(part 1 of 3)
# Autodesk Inventor assembly: coil_driver
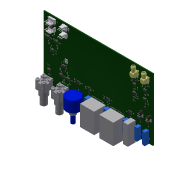
[picture p0: Inventor's stored thumbnail of the model, 180x180]
Saved by Autodesk Inventor 2017 (Build 210142000, 142)
## iProperties
Created: 2017-05-08
Part Number: coil_driver
Description: Component Model
Document SubType Name: Assembly
Designer: nfitch
Authority: Unknown
Sending System: Component
Preprocessor: Open CASCADE STEP processor 6.8
Title: C:/3D/sessions/PPP59106447bd5df/3d/Component/step_file.step
Author: Author
## Documents named in this file (964)
- C:\Users\nfitch\Desktop\repos\Imperial\CCMCircuits\CCM_0008_Coil_Driver\cad\coil_driver.iam
- C:\Users\nfitch\Desktop\repos\Imperial\CCMCircuits\CCM_0008_Coil_Driver\cad\RESC1608X056.ipt
- C:\Users\nfitch\Desktop\repos\Imperial\CCMCircuits\CCM_0008_Coil_Driver\cad\RESC1608X059.ipt
- C:\Users\nfitch\Desktop\repos\Imperial\CCMCircuits\CCM_0008_Coil_Driver\cad\RESC1608X057.ipt
- C:\Users\nfitch\Desktop\repos\Imperial\CCMCircuits\CCM_0008_Coil_Driver\cad\RESC1608X058.ipt
- C:\Users\nfitch\Desktop\repos\Imperial\CCMCircuits\CCM_0008_Coil_Driver\cad\RESC1608X55.ipt
- C:\Users\nfitch\Desktop\repos\Imperial\CCMCircuits\CCM_0008_Coil_Driver\cad\RESC1608X060.ipt
- C:\Users\nfitch\Desktop\repos\Imperial\CCMCircuits\CCM_0008_Coil_Driver\cad\RESC1608X061.ipt
- C:\Users\nfitch\Desktop\repos\Imperial\CCMCircuits\CCM_0008_Coil_Driver\cad\RESC1608X062.ipt
- C:\Users\nfitch\Desktop\repos\Imperial\CCMCircuits\CCM_0008_Coil_Driver\cad\RESC1608X063.ipt
- C:\Users\nfitch\Desktop\repos\Imperial\CCMCircuits\CCM_0008_Coil_Driver\cad\RESC1608X064.ipt
- C:\Users\nfitch\Desktop\repos\Imperial\CCMCircuits\CCM_0008_Coil_Driver\cad\RESC1608X065.ipt
- C:\Users\nfitch\Desktop\repos\Imperial\CCMCircuits\CCM_0008_Coil_Driver\cad\RESC1608X066.ipt
- C:\Users\nfitch\Desktop\repos\Imperial\CCMCircuits\CCM_0008_Coil_Driver\cad\RESC1608X067.ipt
- C:\Users\nfitch\Desktop\repos\Imperial\CCMCircuits\CCM_0008_Coil_Driver\cad\RESC1608X068.ipt
- C:\Users\nfitch\Desktop\repos\Imperial\CCMCircuits\CCM_0008_Coil_Driver\cad\RESC1608X069.ipt
- C:\Users\nfitch\Desktop\repos\Imperial\CCMCircuits\CCM_0008_Coil_Driver\cad\RESC1608X070.ipt
- C:\Users\nfitch\Desktop\repos\Imperial\CCMCircuits\CCM_0008_Coil_Driver\cad\RESC1608X071.ipt
- C:\Users\nfitch\Desktop\repos\Imperial\CCMCircuits\CCM_0008_Coil_Driver\cad\RESC1608X072.ipt
- C:\Users\nfitch\Desktop\repos\Imperial\CCMCircuits\CCM_0008_Coil_Driver\cad\RESC1608X073.ipt
- C:\Users\nfitch\Desktop\repos\Imperial\CCMCircuits\CCM_0008_Coil_Driver\cad\RESC1608X074.ipt
- C:\Users\nfitch\Desktop\repos\Imperial\CCMCircuits\CCM_0008_Coil_Driver\cad\RESC1608X075.ipt
- C:\Users\nfitch\Desktop\repos\Imperial\CCMCircuits\CCM_0008_Coil_Driver\cad\RESC1608X076.ipt
- C:\Users\nfitch\Desktop\repos\Imperial\CCMCircuits\CCM_0008_Coil_Driver\cad\RESC1608X077.ipt
- C:\Users\nfitch\Desktop\repos\Imperial\CCMCircuits\CCM_0008_Coil_Driver\cad\RESC1608X078.ipt
- C:\Users\nfitch\Desktop\repos\Imperial\CCMCircuits\CCM_0008_Coil_Driver\cad\RESC1608X079.ipt
- C:\Users\nfitch\Desktop\repos\Imperial\CCMCircuits\CCM_0008_Coil_Driver\cad\RESC1608X080.ipt
- C:\Users\nfitch\Desktop\repos\Imperial\CCMCircuits\CCM_0008_Coil_Driver\cad\RESC1608X081.ipt
- C:\Users\nfitch\Desktop\repos\Imperial\CCMCircuits\CCM_0008_Coil_Driver\cad\RESC1608X082.ipt
- C:\Users\nfitch\Desktop\repos\Imperial\CCMCircuits\CCM_0008_Coil_Driver\cad\RESC1608X083.ipt
- C:\Users\nfitch\Desktop\repos\Imperial\CCMCircuits\CCM_0008_Coil_Driver\cad\RESC1608X084.ipt
- C:\Users\nfitch\Desktop\repos\Imperial\CCMCircuits\CCM_0008_Coil_Driver\cad\RESC1608X085.ipt
- C:\Users\nfitch\Desktop\repos\Imperial\CCMCircuits\CCM_0008_Coil_Driver\cad\RESC1608X086.ipt
- C:\Users\nfitch\Desktop\repos\Imperial\CCMCircuits\CCM_0008_Coil_Driver\cad\RESC1608X087.ipt
- C:\Users\nfitch\Desktop\repos\Imperial\CCMCircuits\CCM_0008_Coil_Driver\cad\RESC1608X088.ipt
- C:\Users\nfitch\Desktop\repos\Imperial\CCMCircuits\CCM_0008_Coil_Driver\cad\RESC1608X089.ipt
- C:\Users\nfitch\Desktop\repos\Imperial\CCMCircuits\CCM_0008_Coil_Driver\cad\RESC1608X090.ipt
- C:\Users\nfitch\Desktop\repos\Imperial\CCMCircuits\CCM_0008_Coil_Driver\cad\RESC1608X091.ipt
- C:\Users\nfitch\Desktop\repos\Imperial\CCMCircuits\CCM_0008_Coil_Driver\cad\RESC1608X092.ipt
- C:\Users\nfitch\Desktop\repos\Imperial\CCMCircuits\CCM_0008_Coil_Driver\cad\RESC1608X093.ipt
- C:\Users\nfitch\Desktop\repos\Imperial\CCMCircuits\CCM_0008_Coil_Driver\cad\RESC1608X094.ipt
- C:\Users\nfitch\Desktop\repos\Imperial\CCMCircuits\CCM_0008_Coil_Driver\cad\RESC1608X095.ipt
- C:\Users\nfitch\Desktop\repos\Imperial\CCMCircuits\CCM_0008_Coil_Driver\cad\RESC1608X096.ipt
- C:\Users\nfitch\Desktop\repos\Imperial\CCMCircuits\CCM_0008_Coil_Driver\cad\RESC1608X097.ipt
- C:\Users\nfitch\Desktop\repos\Imperial\CCMCircuits\CCM_0008_Coil_Driver\cad\RESC1608X098.ipt
- C:\Users\nfitch\Desktop\repos\Imperial\CCMCircuits\CCM_0008_Coil_Driver\cad\RESC1608X099.ipt
- C:\Users\nfitch\Desktop\repos\Imperial\CCMCircuits\CCM_0008_Coil_Driver\cad\RESC1608X100.ipt
- C:\Users\nfitch\Desktop\repos\Imperial\CCMCircuits\CCM_0008_Coil_Driver\cad\RESC1608X101.ipt
- C:\Users\nfitch\Desktop\repos\Imperial\CCMCircuits\CCM_0008_Coil_Driver\cad\RESC1608X102.ipt
- C:\Users\nfitch\Desktop\repos\Imperial\CCMCircuits\CCM_0008_Coil_Driver\cad\RESC1608X103.ipt
- C:\Users\nfitch\Desktop\repos\Imperial\CCMCircuits\CCM_0008_Coil_Driver\cad\RESC1608X104.ipt
- C:\Users\nfitch\Desktop\repos\Imperial\CCMCircuits\CCM_0008_Coil_Driver\cad\RESC1608X105.ipt
- C:\Users\nfitch\Desktop\repos\Imperial\CCMCircuits\CCM_0008_Coil_Driver\cad\RESC1608X106.ipt
- C:\Users\nfitch\Desktop\repos\Imperial\CCMCircuits\CCM_0008_Coil_Driver\cad\RESC1608X107.ipt
- C:\Users\nfitch\Desktop\repos\Imperial\CCMCircuits\CCM_0008_Coil_Driver\cad\RESC1608X108.ipt
- C:\Users\nfitch\Desktop\repos\Imperial\CCMCircuits\CCM_0008_Coil_Driver\cad\RESC1608X109.ipt
- C:\Users\nfitch\Desktop\repos\Imperial\CCMCircuits\CCM_0008_Coil_Driver\cad\RESC1608X110.ipt
- C:\Users\nfitch\Desktop\repos\Imperial\CCMCircuits\CCM_0008_Coil_Driver\cad\RESC1608X111.ipt
- C:\Users\nfitch\Desktop\repos\Imperial\CCMCircuits\CCM_0008_Coil_Driver\cad\RESC1608X112.ipt
- C:\Users\nfitch\Desktop\repos\Imperial\CCMCircuits\CCM_0008_Coil_Driver\cad\RESC1608X113.ipt
- C:\Users\nfitch\Desktop\repos\Imperial\CCMCircuits\CCM_0008_Coil_Driver\cad\RESC1608X114.ipt
- C:\Users\nfitch\Desktop\repos\Imperial\CCMCircuits\CCM_0008_Coil_Driver\cad\RESC1608X115.ipt
- C:\Users\nfitch\Desktop\repos\Imperial\CCMCircuits\CCM_0008_Coil_Driver\cad\RESC1608X116.ipt
- C:\Users\nfitch\Desktop\repos\Imperial\CCMCircuits\CCM_0008_Coil_Driver\cad\RESC1608X117.ipt
- C:\Users\nfitch\Desktop\repos\Imperial\CCMCircuits\CCM_0008_Coil_Driver\cad\RESC1608X118.ipt
- C:\Users\nfitch\Desktop\repos\Imperial\CCMCircuits\CCM_0008_Coil_Driver\cad\RESC1608X119.ipt
- C:\Users\nfitch\Desktop\repos\Imperial\CCMCircuits\CCM_0008_Coil_Driver\cad\RESC1608X120.ipt
- C:\Users\nfitch\Desktop\repos\Imperial\CCMCircuits\CCM_0008_Coil_Driver\cad\RESC1608X121.ipt
- C:\Users\nfitch\Desktop\repos\Imperial\CCMCircuits\CCM_0008_Coil_Driver\cad\RESC1608X122.ipt
- C:\Users\nfitch\Desktop\repos\Imperial\CCMCircuits\CCM_0008_Coil_Driver\cad\RESC1608X123.ipt
- C:\Users\nfitch\Desktop\repos\Imperial\CCMCircuits\CCM_0008_Coil_Driver\cad\RESC1608X124.ipt
- C:\Users\nfitch\Desktop\repos\Imperial\CCMCircuits\CCM_0008_Coil_Driver\cad\RESC1608X125.ipt
- C:\Users\nfitch\Desktop\repos\Imperial\CCMCircuits\CCM_0008_Coil_Driver\cad\RESC1608X126.ipt
- C:\Users\nfitch\Desktop\repos\Imperial\CCMCircuits\CCM_0008_Coil_Driver\cad\RESC1608X127.ipt
- C:\Users\nfitch\Desktop\repos\Imperial\CCMCircuits\CCM_0008_Coil_Driver\cad\RESC1608X128.ipt
- C:\Users\nfitch\Desktop\repos\Imperial\CCMCircuits\CCM_0008_Coil_Driver\cad\RESC1608X129.ipt
- C:\Users\nfitch\Desktop\repos\Imperial\CCMCircuits\CCM_0008_Coil_Driver\cad\RESC1608X130.ipt
- C:\Users\nfitch\Desktop\repos\Imperial\CCMCircuits\CCM_0008_Coil_Driver\cad\RESC1608X131.ipt
- C:\Users\nfitch\Desktop\repos\Imperial\CCMCircuits\CCM_0008_Coil_Driver\cad\RESC1608X132.ipt
- C:\Users\nfitch\Desktop\repos\Imperial\CCMCircuits\CCM_0008_Coil_Driver\cad\RESC1608X133.ipt
- C:\Users\nfitch\Desktop\repos\Imperial\CCMCircuits\CCM_0008_Coil_Driver\cad\RESC1608X134.ipt
- C:\Users\nfitch\Desktop\repos\Imperial\CCMCircuits\CCM_0008_Coil_Driver\cad\RESC1608X135.ipt
- C:\Users\nfitch\Desktop\repos\Imperial\CCMCircuits\CCM_0008_Coil_Driver\cad\RESC1608X136.ipt
- C:\Users\nfitch\Desktop\repos\Imperial\CCMCircuits\CCM_0008_Coil_Driver\cad\RESC1608X137.ipt
- C:\Users\nfitch\Desktop\repos\Imperial\CCMCircuits\CCM_0008_Coil_Driver\cad\RESC1608X138.ipt
- C:\Users\nfitch\Desktop\repos\Imperial\CCMCircuits\CCM_0008_Coil_Driver\cad\RESC1608X139.ipt
- C:\Users\nfitch\Desktop\repos\Imperial\CCMCircuits\CCM_0008_Coil_Driver\cad\RESC1608X140.ipt
- C:\Users\nfitch\Desktop\repos\Imperial\CCMCircuits\CCM_0008_Coil_Driver\cad\RESC1608X141.ipt
- C:\Users\nfitch\Desktop\repos\Imperial\CCMCircuits\CCM_0008_Coil_Driver\cad\RESC1608X142.ipt
- C:\Users\nfitch\Desktop\repos\Imperial\CCMCircuits\CCM_0008_Coil_Driver\cad\RESC1608X143.ipt
- C:\Users\nfitch\Desktop\repos\Imperial\CCMCircuits\CCM_0008_Coil_Driver\cad\RESC1608X144.ipt
- C:\Users\nfitch\Desktop\repos\Imperial\CCMCircuits\CCM_0008_Coil_Driver\cad\RESC1608X145.ipt
- C:\Users\nfitch\Desktop\repos\Imperial\CCMCircuits\CCM_0008_Coil_Driver\cad\RESC1608X146.ipt
- C:\Users\nfitch\Desktop\repos\Imperial\CCMCircuits\CCM_0008_Coil_Driver\cad\RESC1608X147.ipt
- C:\Users\nfitch\Desktop\repos\Imperial\CCMCircuits\CCM_0008_Coil_Driver\cad\RESC1608X148.ipt
- C:\Users\nfitch\Desktop\repos\Imperial\CCMCircuits\CCM_0008_Coil_Driver\cad\RESC1608X149.ipt
- C:\Users\nfitch\Desktop\repos\Imperial\CCMCircuits\CCM_0008_Coil_Driver\cad\RESC1608X150.ipt
- C:\Users\nfitch\Desktop\repos\Imperial\CCMCircuits\CCM_0008_Coil_Driver\cad\RESC1608X151.ipt
- C:\Users\nfitch\Desktop\repos\Imperial\CCMCircuits\CCM_0008_Coil_Driver\cad\RESC1608X152.ipt
- C:\Users\nfitch\Desktop\repos\Imperial\CCMCircuits\CCM_0008_Coil_Driver\cad\RESC1608X153.ipt
- C:\Users\nfitch\Desktop\repos\Imperial\CCMCircuits\CCM_0008_Coil_Driver\cad\RESC1608X154.ipt
- C:\Users\nfitch\Desktop\repos\Imperial\CCMCircuits\CCM_0008_Coil_Driver\cad\RESC1608X155.ipt
- C:\Users\nfitch\Desktop\repos\Imperial\CCMCircuits\CCM_0008_Coil_Driver\cad\RESC1608X156.ipt
- C:\Users\nfitch\Desktop\repos\Imperial\CCMCircuits\CCM_0008_Coil_Driver\cad\RESC1608X157.ipt
- C:\Users\nfitch\Desktop\repos\Imperial\CCMCircuits\CCM_0008_Coil_Driver\cad\RESC1608X158.ipt
- C:\Users\nfitch\Desktop\repos\Imperial\CCMCircuits\CCM_0008_Coil_Driver\cad\RESC1608X159.ipt
- C:\Users\nfitch\Desktop\repos\Imperial\CCMCircuits\CCM_0008_Coil_Driver\cad\RESC1608X160.ipt
- C:\Users\nfitch\Desktop\repos\Imperial\CCMCircuits\CCM_0008_Coil_Driver\cad\RESC1608X161.ipt
- C:\Users\nfitch\Desktop\repos\Imperial\CCMCircuits\CCM_0008_Coil_Driver\cad\RESC1608X162.ipt
- C:\Users\nfitch\Desktop\repos\Imperial\CCMCircuits\CCM_0008_Coil_Driver\cad\RESC1608X163.ipt
- C:\Users\nfitch\Desktop\repos\Imperial\CCMCircuits\CCM_0008_Coil_Driver\cad\RESC1608X164.ipt
- C:\Users\nfitch\Desktop\repos\Imperial\CCMCircuits\CCM_0008_Coil_Driver\cad\RESC1608X165.ipt
- C:\Users\nfitch\Desktop\repos\Imperial\CCMCircuits\CCM_0008_Coil_Driver\cad\RESC1608X166.ipt
- C:\Users\nfitch\Desktop\repos\Imperial\CCMCircuits\CCM_0008_Coil_Driver\cad\RESC1608X167.ipt
- C:\Users\nfitch\Desktop\repos\Imperial\CCMCircuits\CCM_0008_Coil_Driver\cad\RESC1608X168.ipt
- C:\Users\nfitch\Desktop\repos\Imperial\CCMCircuits\CCM_0008_Coil_Driver\cad\RESC1608X169.ipt
- C:\Users\nfitch\Desktop\repos\Imperial\CCMCircuits\CCM_0008_Coil_Driver\cad\RESC1608X170.ipt
- C:\Users\nfitch\Desktop\repos\Imperial\CCMCircuits\CCM_0008_Coil_Driver\cad\RESC1608X171.ipt
- C:\Users\nfitch\Desktop\repos\Imperial\CCMCircuits\CCM_0008_Coil_Driver\cad\RESC1608X172.ipt
- C:\Users\nfitch\Desktop\repos\Imperial\CCMCircuits\CCM_0008_Coil_Driver\cad\RESC1608X173.ipt
- C:\Users\nfitch\Desktop\repos\Imperial\CCMCircuits\CCM_0008_Coil_Driver\cad\RESC1608X174.ipt
- C:\Users\nfitch\Desktop\repos\Imperial\CCMCircuits\CCM_0008_Coil_Driver\cad\RESC1608X175.ipt
- C:\Users\nfitch\Desktop\repos\Imperial\CCMCircuits\CCM_0008_Coil_Driver\cad\RESC1608X176.ipt
- C:\Users\nfitch\Desktop\repos\Imperial\CCMCircuits\CCM_0008_Coil_Driver\cad\RESC1608X177.ipt
- C:\Users\nfitch\Desktop\repos\Imperial\CCMCircuits\CCM_0008_Coil_Driver\cad\RESC1608X178.ipt
- C:\Users\nfitch\Desktop\repos\Imperial\CCMCircuits\CCM_0008_Coil_Driver\cad\RESC1608X179.ipt
- C:\Users\nfitch\Desktop\repos\Imperial\CCMCircuits\CCM_0008_Coil_Driver\cad\RESC1608X180.ipt
- C:\Users\nfitch\Desktop\repos\Imperial\CCMCircuits\CCM_0008_Coil_Driver\cad\RESC1608X181.ipt
- C:\Users\nfitch\Desktop\repos\Imperial\CCMCircuits\CCM_0008_Coil_Driver\cad\RESC1608X182.ipt
- C:\Users\nfitch\Desktop\repos\Imperial\CCMCircuits\CCM_0008_Coil_Driver\cad\RESC1608X183.ipt
- C:\Users\nfitch\Desktop\repos\Imperial\CCMCircuits\CCM_0008_Coil_Driver\cad\RESC1608X184.ipt
- C:\Users\nfitch\Desktop\repos\Imperial\CCMCircuits\CCM_0008_Coil_Driver\cad\RESC1608X185.ipt
- C:\Users\nfitch\Desktop\repos\Imperial\CCMCircuits\CCM_0008_Coil_Driver\cad\RESC1608X186.ipt
- C:\Users\nfitch\Desktop\repos\Imperial\CCMCircuits\CCM_0008_Coil_Driver\cad\RESC1608X187.ipt
- C:\Users\nfitch\Desktop\repos\Imperial\CCMCircuits\CCM_0008_Coil_Driver\cad\RESC1608X188.ipt
- C:\Users\nfitch\Desktop\repos\Imperial\CCMCircuits\CCM_0008_Coil_Driver\cad\RESC1608X189.ipt
- C:\Users\nfitch\Desktop\repos\Imperial\CCMCircuits\CCM_0008_Coil_Driver\cad\RESC1608X190.ipt
- C:\Users\nfitch\Desktop\repos\Imperial\CCMCircuits\CCM_0008_Coil_Driver\cad\RESC1608X191.ipt
- C:\Users\nfitch\Desktop\repos\Imperial\CCMCircuits\CCM_0008_Coil_Driver\cad\RESC1608X192.ipt
- C:\Users\nfitch\Desktop\repos\Imperial\CCMCircuits\CCM_0008_Coil_Driver\cad\RESC1608X193.ipt
- C:\Users\nfitch\Desktop\repos\Imperial\CCMCircuits\CCM_0008_Coil_Driver\cad\RESC1608X194.ipt
- C:\Users\nfitch\Desktop\repos\Imperial\CCMCircuits\CCM_0008_Coil_Driver\cad\RESC1608X195.ipt
- C:\Users\nfitch\Desktop\repos\Imperial\CCMCircuits\CCM_0008_Coil_Driver\cad\RESC1608X196.ipt
- C:\Users\nfitch\Desktop\repos\Imperial\CCMCircuits\CCM_0008_Coil_Driver\cad\RESC1608X197.ipt
- C:\Users\nfitch\Desktop\repos\Imperial\CCMCircuits\CCM_0008_Coil_Driver\cad\RESC1608X198.ipt
- C:\Users\nfitch\Desktop\repos\Imperial\CCMCircuits\CCM_0008_Coil_Driver\cad\RESC1608X199.ipt
- C:\Users\nfitch\Desktop\repos\Imperial\CCMCircuits\CCM_0008_Coil_Driver\cad\RESC1608X200.ipt
- C:\Users\nfitch\Desktop\repos\Imperial\CCMCircuits\CCM_0008_Coil_Driver\cad\RESC1608X201.ipt
- C:\Users\nfitch\Desktop\repos\Imperial\CCMCircuits\CCM_0008_Coil_Driver\cad\RESC1608X202.ipt
- C:\Users\nfitch\Desktop\repos\Imperial\CCMCircuits\CCM_0008_Coil_Driver\cad\RESC1608X203.ipt
- C:\Users\nfitch\Desktop\repos\Imperial\CCMCircuits\CCM_0008_Coil_Driver\cad\RESC1608X204.ipt
- C:\Users\nfitch\Desktop\repos\Imperial\CCMCircuits\CCM_0008_Coil_Driver\cad\RESC1608X205.ipt
- C:\Users\nfitch\Desktop\repos\Imperial\CCMCircuits\CCM_0008_Coil_Driver\cad\RESC1608X206.ipt
- C:\Users\nfitch\Desktop\repos\Imperial\CCMCircuits\CCM_0008_Coil_Driver\cad\RESC1608X207.ipt
- C:\Users\nfitch\Desktop\repos\Imperial\CCMCircuits\CCM_0008_Coil_Driver\cad\RESC1608X208.ipt
- C:\Users\nfitch\Desktop\repos\Imperial\CCMCircuits\CCM_0008_Coil_Driver\cad\RESC1608X209.ipt
- C:\Users\nfitch\Desktop\repos\Imperial\CCMCircuits\CCM_0008_Coil_Driver\cad\RESC1608X210.ipt
- C:\Users\nfitch\Desktop\repos\Imperial\CCMCircuits\CCM_0008_Coil_Driver\cad\RESC1608X211.ipt
- C:\Users\nfitch\Desktop\repos\Imperial\CCMCircuits\CCM_0008_Coil_Driver\cad\RESC1608X212.ipt
- C:\Users\nfitch\Desktop\repos\Imperial\CCMCircuits\CCM_0008_Coil_Driver\cad\RESC1608X213.ipt
- C:\Users\nfitch\Desktop\repos\Imperial\CCMCircuits\CCM_0008_Coil_Driver\cad\RESC1608X214.ipt
- C:\Users\nfitch\Desktop\repos\Imperial\CCMCircuits\CCM_0008_Coil_Driver\cad\RESC1608X215.ipt
- C:\Users\nfitch\Desktop\repos\Imperial\CCMCircuits\CCM_0008_Coil_Driver\cad\RESC1608X216.ipt
- C:\Users\nfitch\Desktop\repos\Imperial\CCMCircuits\CCM_0008_Coil_Driver\cad\RESC1608X217.ipt
- C:\Users\nfitch\Desktop\repos\Imperial\CCMCircuits\CCM_0008_Coil_Driver\cad\RESC1608X218.ipt
- C:\Users\nfitch\Desktop\repos\Imperial\CCMCircuits\CCM_0008_Coil_Driver\cad\RESC1608X219.ipt
- C:\Users\nfitch\Desktop\repos\Imperial\CCMCircuits\CCM_0008_Coil_Driver\cad\RESC1608X220.ipt
- C:\Users\nfitch\Desktop\repos\Imperial\CCMCircuits\CCM_0008_Coil_Driver\cad\RESC1608X221.ipt
- C:\Users\nfitch\Desktop\repos\Imperial\CCMCircuits\CCM_0008_Coil_Driver\cad\RESC1608X222.ipt
- C:\Users\nfitch\Desktop\repos\Imperial\CCMCircuits\CCM_0008_Coil_Driver\cad\RESC1608X223.ipt
- C:\Users\nfitch\Desktop\repos\Imperial\CCMCircuits\CCM_0008_Coil_Driver\cad\RESC1608X224.ipt
- C:\Users\nfitch\Desktop\repos\Imperial\CCMCircuits\CCM_0008_Coil_Driver\cad\RESC1608X225.ipt
- C:\Users\nfitch\Desktop\repos\Imperial\CCMCircuits\CCM_0008_Coil_Driver\cad\RESC1608X226.ipt
- C:\Users\nfitch\Desktop\repos\Imperial\CCMCircuits\CCM_0008_Coil_Driver\cad\RESC1608X227.ipt
- C:\Users\nfitch\Desktop\repos\Imperial\CCMCircuits\CCM_0008_Coil_Driver\cad\RESC1608X228.ipt
- C:\Users\nfitch\Desktop\repos\Imperial\CCMCircuits\CCM_0008_Coil_Driver\cad\RESC1608X229.ipt
- C:\Users\nfitch\Desktop\repos\Imperial\CCMCircuits\CCM_0008_Coil_Driver\cad\RESC1608X230.ipt
- C:\Users\nfitch\Desktop\repos\Imperial\CCMCircuits\CCM_0008_Coil_Driver\cad\RESC1608X231.ipt
- C:\Users\nfitch\Desktop\repos\Imperial\CCMCircuits\CCM_0008_Coil_Driver\cad\RESC1608X232.ipt
- C:\Users\nfitch\Desktop\repos\Imperial\CCMCircuits\CCM_0008_Coil_Driver\cad\RESC1608X233.ipt
- C:\Users\nfitch\Desktop\repos\Imperial\CCMCircuits\CCM_0008_Coil_Driver\cad\RESC1608X234.ipt
- C:\Users\nfitch\Desktop\repos\Imperial\CCMCircuits\CCM_0008_Coil_Driver\cad\RESC1608X235.ipt
- C:\Users\nfitch\Desktop\repos\Imperial\CCMCircuits\CCM_0008_Coil_Driver\cad\RESC1608X236.ipt
- C:\Users\nfitch\Desktop\repos\Imperial\CCMCircuits\CCM_0008_Coil_Driver\cad\RESC1608X237.ipt
- C:\Users\nfitch\Desktop\repos\Imperial\CCMCircuits\CCM_0008_Coil_Driver\cad\RESC1608X238.ipt
- C:\Users\nfitch\Desktop\repos\Imperial\CCMCircuits\CCM_0008_Coil_Driver\cad\RESC1608X239.ipt
- C:\Users\nfitch\Desktop\repos\Imperial\CCMCircuits\CCM_0008_Coil_Driver\cad\RESC1608X240.ipt
- C:\Users\nfitch\Desktop\repos\Imperial\CCMCircuits\CCM_0008_Coil_Driver\cad\RESC1608X241.ipt
- C:\Users\nfitch\Desktop\repos\Imperial\CCMCircuits\CCM_0008_Coil_Driver\cad\RESC1608X242.ipt
- C:\Users\nfitch\Desktop\repos\Imperial\CCMCircuits\CCM_0008_Coil_Driver\cad\RESC1608X243.ipt
- C:\Users\nfitch\Desktop\repos\Imperial\CCMCircuits\CCM_0008_Coil_Driver\cad\RESC1608X244.ipt
- C:\Users\nfitch\Desktop\repos\Imperial\CCMCircuits\CCM_0008_Coil_Driver\cad\RESC1608X245.ipt
- C:\Users\nfitch\Desktop\repos\Imperial\CCMCircuits\CCM_0008_Coil_Driver\cad\RESC1608X246.ipt
- C:\Users\nfitch\Desktop\repos\Imperial\CCMCircuits\CCM_0008_Coil_Driver\cad\RESC1608X247.ipt
- C:\Users\nfitch\Desktop\repos\Imperial\CCMCircuits\CCM_0008_Coil_Driver\cad\RESC1608X248.ipt
- C:\Users\nfitch\Desktop\repos\Imperial\CCMCircuits\CCM_0008_Coil_Driver\cad\RESC1608X249.ipt
- C:\Users\nfitch\Desktop\repos\Imperial\CCMCircuits\CCM_0008_Coil_Driver\cad\RESC1608X250.ipt
- C:\Users\nfitch\Desktop\repos\Imperial\CCMCircuits\CCM_0008_Coil_Driver\cad\RESC1608X251.ipt
- C:\Users\nfitch\Desktop\repos\Imperial\CCMCircuits\CCM_0008_Coil_Driver\cad\RESC1608X252.ipt
- C:\Users\nfitch\Desktop\repos\Imperial\CCMCircuits\CCM_0008_Coil_Driver\cad\RESC1608X253.ipt
- C:\Users\nfitch\Desktop\repos\Imperial\CCMCircuits\CCM_0008_Coil_Driver\cad\RESC1608X254.ipt
- C:\Users\nfitch\Desktop\repos\Imperial\CCMCircuits\CCM_0008_Coil_Driver\cad\RESC1608X255.ipt
- C:\Users\nfitch\Desktop\repos\Imperial\CCMCircuits\CCM_0008_Coil_Driver\cad\RESC1608X256.ipt
- C:\Users\nfitch\Desktop\repos\Imperial\CCMCircuits\CCM_0008_Coil_Driver\cad\RESC1608X257.ipt
- C:\Users\nfitch\Desktop\repos\Imperial\CCMCircuits\CCM_0008_Coil_Driver\cad\RESC1608X258.ipt
- C:\Users\nfitch\Desktop\repos\Imperial\CCMCircuits\CCM_0008_Coil_Driver\cad\RESC1608X259.ipt
- C:\Users\nfitch\Desktop\repos\Imperial\CCMCircuits\CCM_0008_Coil_Driver\cad\RESC1608X260.ipt
- C:\Users\nfitch\Desktop\repos\Imperial\CCMCircuits\CCM_0008_Coil_Driver\cad\RESC1608X261.ipt
- C:\Users\nfitch\Desktop\repos\Imperial\CCMCircuits\CCM_0008_Coil_Driver\cad\RESC1608X262.ipt
- C:\Users\nfitch\Desktop\repos\Imperial\CCMCircuits\CCM_0008_Coil_Driver\cad\RESC1608X263.ipt
- C:\Users\nfitch\Desktop\repos\Imperial\CCMCircuits\CCM_0008_Coil_Driver\cad\RESC1608X264.ipt
- C:\Users\nfitch\Desktop\repos\Imperial\CCMCircuits\CCM_0008_Coil_Driver\cad\RESC1608X265.ipt
- C:\Users\nfitch\Desktop\repos\Imperial\CCMCircuits\CCM_0008_Coil_Driver\cad\RESC1608X266.ipt
- C:\Users\nfitch\Desktop\repos\Imperial\CCMCircuits\CCM_0008_Coil_Driver\cad\RESC1608X267.ipt
- C:\Users\nfitch\Desktop\repos\Imperial\CCMCircuits\CCM_0008_Coil_Driver\cad\RESC1608X268.ipt
- C:\Users\nfitch\Desktop\repos\Imperial\CCMCircuits\CCM_0008_Coil_Driver\cad\RESC1608X269.ipt
- C:\Users\nfitch\Desktop\repos\Imperial\CCMCircuits\CCM_0008_Coil_Driver\cad\RESC1608X270.ipt
- C:\Users\nfitch\Desktop\repos\Imperial\CCMCircuits\CCM_0008_Coil_Driver\cad\RESC1608X271.ipt
- C:\Users\nfitch\Desktop\repos\Imperial\CCMCircuits\CCM_0008_Coil_Driver\cad\RESC1608X272.ipt
- C:\Users\nfitch\Desktop\repos\Imperial\CCMCircuits\CCM_0008_Coil_Driver\cad\RESC1608X273.ipt
- C:\Users\nfitch\Desktop\repos\Imperial\CCMCircuits\CCM_0008_Coil_Driver\cad\RESC1608X274.ipt
- C:\Users\nfitch\Desktop\repos\Imperial\CCMCircuits\CCM_0008_Coil_Driver\cad\RESC1608X275.ipt
- C:\Users\nfitch\Desktop\repos\Imperial\CCMCircuits\CCM_0008_Coil_Driver\cad\RESC1608X276.ipt
- C:\Users\nfitch\Desktop\repos\Imperial\CCMCircuits\CCM_0008_Coil_Driver\cad\RESC1608X277.ipt
- C:\Users\nfitch\Desktop\repos\Imperial\CCMCircuits\CCM_0008_Coil_Driver\cad\RESC1608X278.ipt
- C:\Users\nfitch\Desktop\repos\Imperial\CCMCircuits\CCM_0008_Coil_Driver\cad\RESC1608X279.ipt
- C:\Users\nfitch\Desktop\repos\Imperial\CCMCircuits\CCM_0008_Coil_Driver\cad\RESC1608X280.ipt
- C:\Users\nfitch\Desktop\repos\Imperial\CCMCircuits\CCM_0008_Coil_Driver\cad\RESC1608X281.ipt
- C:\Users\nfitch\Desktop\repos\Imperial\CCMCircuits\CCM_0008_Coil_Driver\cad\RESC1608X282.ipt
- C:\Users\nfitch\Desktop\repos\Imperial\CCMCircuits\CCM_0008_Coil_Driver\cad\RESC1608X283.ipt
- C:\Users\nfitch\Desktop\repos\Imperial\CCMCircuits\CCM_0008_Coil_Driver\cad\RESC1608X284.ipt
- C:\Users\nfitch\Desktop\repos\Imperial\CCMCircuits\CCM_0008_Coil_Driver\cad\RESC1608X285.ipt
- C:\Users\nfitch\Desktop\repos\Imperial\CCMCircuits\CCM_0008_Coil_Driver\cad\RESC1608X286.ipt
- C:\Users\nfitch\Desktop\repos\Imperial\CCMCircuits\CCM_0008_Coil_Driver\cad\RESC1608X287.ipt
- C:\Users\nfitch\Desktop\repos\Imperial\CCMCircuits\CCM_0008_Coil_Driver\cad\RESC1608X288.ipt
- C:\Users\nfitch\Desktop\repos\Imperial\CCMCircuits\CCM_0008_Coil_Driver\cad\RESC1608X289.ipt
- C:\Users\nfitch\Desktop\repos\Imperial\CCMCircuits\CCM_0008_Coil_Driver\cad\RESC1608X290.ipt
- C:\Users\nfitch\Desktop\repos\Imperial\CCMCircuits\CCM_0008_Coil_Driver\cad\RESC1608X291.ipt
- C:\Users\nfitch\Desktop\repos\Imperial\CCMCircuits\CCM_0008_Coil_Driver\cad\RESC1608X292.ipt
- C:\Users\nfitch\Desktop\repos\Imperial\CCMCircuits\CCM_0008_Coil_Driver\cad\RESC1608X293.ipt
- C:\Users\nfitch\Desktop\repos\Imperial\CCMCircuits\CCM_0008_Coil_Driver\cad\RESC1608X294.ipt
- C:\Users\nfitch\Desktop\repos\Imperial\CCMCircuits\CCM_0008_Coil_Driver\cad\RESC1608X295.ipt
- C:\Users\nfitch\Desktop\repos\Imperial\CCMCircuits\CCM_0008_Coil_Driver\cad\RESC1608X296.ipt
- C:\Users\nfitch\Desktop\repos\Imperial\CCMCircuits\CCM_0008_Coil_Driver\cad\RESC1608X297.ipt
- C:\Users\nfitch\Desktop\repos\Imperial\CCMCircuits\CCM_0008_Coil_Driver\cad\RESC1608X298.ipt
- C:\Users\nfitch\Desktop\repos\Imperial\CCMCircuits\CCM_0008_Coil_Driver\cad\RESC1608X299.ipt
- C:\Users\nfitch\Desktop\repos\Imperial\CCMCircuits\CCM_0008_Coil_Driver\cad\RESC1608X300.ipt
- C:\Users\nfitch\Desktop\repos\Imperial\CCMCircuits\CCM_0008_Coil_Driver\cad\RESC1608X301.ipt
- C:\Users\nfitch\Desktop\repos\Imperial\CCMCircuits\CCM_0008_Coil_Driver\cad\RESC1608X302.ipt
- C:\Users\nfitch\Desktop\repos\Imperial\CCMCircuits\CCM_0008_Coil_Driver\cad\RESC1608X303.ipt
- C:\Users\nfitch\Desktop\repos\Imperial\CCMCircuits\CCM_0008_Coil_Driver\cad\RESC1608X304.ipt
- C:\Users\nfitch\Desktop\repos\Imperial\CCMCircuits\CCM_0008_Coil_Driver\cad\RESC1608X305.ipt
- C:\Users\nfitch\Desktop\repos\Imperial\CCMCircuits\CCM_0008_Coil_Driver\cad\RESC1608X306.ipt
- C:\Users\nfitch\Desktop\repos\Imperial\CCMCircuits\CCM_0008_Coil_Driver\cad\RESC1608X307.ipt
- C:\Users\nfitch\Desktop\repos\Imperial\CCMCircuits\CCM_0008_Coil_Driver\cad\RESC1608X308.ipt
- C:\Users\nfitch\Desktop\repos\Imperial\CCMCircuits\CCM_0008_Coil_Driver\cad\RESC1608X309.ipt
- C:\Users\nfitch\Desktop\repos\Imperial\CCMCircuits\CCM_0008_Coil_Driver\cad\RESC1608X310.ipt
- C:\Users\nfitch\Desktop\repos\Imperial\CCMCircuits\CCM_0008_Coil_Driver\cad\RESC1608X311.ipt
- C:\Users\nfitch\Desktop\repos\Imperial\CCMCircuits\CCM_0008_Coil_Driver\cad\RESC1608X312.ipt
- C:\Users\nfitch\Desktop\repos\Imperial\CCMCircuits\CCM_0008_Coil_Driver\cad\RESC1608X313.ipt
- C:\Users\nfitch\Desktop\repos\Imperial\CCMCircuits\CCM_0008_Coil_Driver\cad\RESC1608X314.ipt
- C:\Users\nfitch\Desktop\repos\Imperial\CCMCircuits\CCM_0008_Coil_Driver\cad\RESC1608X315.ipt
- C:\Users\nfitch\Desktop\repos\Imperial\CCMCircuits\CCM_0008_Coil_Driver\cad\RESC1608X316.ipt
- C:\Users\nfitch\Desktop\repos\Imperial\CCMCircuits\CCM_0008_Coil_Driver\cad\RESC1608X317.ipt
- C:\Users\nfitch\Desktop\repos\Imperial\CCMCircuits\CCM_0008_Coil_Driver\cad\RESC1608X318.ipt
- C:\Users\nfitch\Desktop\repos\Imperial\CCMCircuits\CCM_0008_Coil_Driver\cad\RESC1608X319.ipt
- C:\Users\nfitch\Desktop\repos\Imperial\CCMCircuits\CCM_0008_Coil_Driver\cad\RESC1608X320.ipt
- C:\Users\nfitch\Desktop\repos\Imperial\CCMCircuits\CCM_0008_Coil_Driver\cad\RESC1608X321.ipt
- C:\Users\nfitch\Desktop\repos\Imperial\CCMCircuits\CCM_0008_Coil_Driver\cad\RESC1608X322.ipt
- C:\Users\nfitch\Desktop\repos\Imperial\CCMCircuits\CCM_0008_Coil_Driver\cad\RESC1608X323.ipt
- C:\Users\nfitch\Desktop\repos\Imperial\CCMCircuits\CCM_0008_Coil_Driver\cad\RESC1608X324.ipt
- C:\Users\nfitch\Desktop\repos\Imperial\CCMCircuits\CCM_0008_Coil_Driver\cad\RESC1608X325.ipt
- C:\Users\nfitch\Desktop\repos\Imperial\CCMCircuits\CCM_0008_Coil_Driver\cad\RESC1608X326.ipt
- C:\Users\nfitch\Desktop\repos\Imperial\CCMCircuits\CCM_0008_Coil_Driver\cad\RESC1608X327.ipt
- C:\Users\nfitch\Desktop\repos\Imperial\CCMCircuits\CCM_0008_Coil_Driver\cad\RESC1608X328.ipt
- C:\Users\nfitch\Desktop\repos\Imperial\CCMCircuits\CCM_0008_Coil_Driver\cad\RESC1608X329.ipt
- C:\Users\nfitch\Desktop\repos\Imperial\CCMCircuits\CCM_0008_Coil_Driver\cad\RESC1608X330.ipt
- C:\Users\nfitch\Desktop\repos\Imperial\CCMCircuits\CCM_0008_Coil_Driver\cad\RESC1608X331.ipt
- C:\Users\nfitch\Desktop\repos\Imperial\CCMCircuits\CCM_0008_Coil_Driver\cad\RESC1608X332.ipt
- C:\Users\nfitch\Desktop\repos\Imperial\CCMCircuits\CCM_0008_Coil_Driver\cad\RESC1608X333.ipt
- C:\Users\nfitch\Desktop\repos\Imperial\CCMCircuits\CCM_0008_Coil_Driver\cad\RESC1608X334.ipt
- C:\Users\nfitch\Desktop\repos\Imperial\CCMCircuits\CCM_0008_Coil_Driver\cad\RESC1608X335.ipt
- C:\Users\nfitch\Desktop\repos\Imperial\CCMCircuits\CCM_0008_Coil_Driver\cad\RESC1608X336.ipt
- C:\Users\nfitch\Desktop\repos\Imperial\CCMCircuits\CCM_0008_Coil_Driver\cad\RESC1608X337.ipt
- C:\Users\nfitch\Desktop\repos\Imperial\CCMCircuits\CCM_0008_Coil_Driver\cad\RESC1608X338.ipt
- C:\Users\nfitch\Desktop\repos\Imperial\CCMCircuits\CCM_0008_Coil_Driver\cad\RESC1608X339.ipt
- C:\Users\nfitch\Desktop\repos\Imperial\CCMCircuits\CCM_0008_Coil_Driver\cad\RESC1608X340.ipt
- C:\Users\nfitch\Desktop\repos\Imperial\CCMCircuits\CCM_0008_Coil_Driver\cad\RESC1608X341.ipt
- C:\Users\nfitch\Desktop\repos\Imperial\CCMCircuits\CCM_0008_Coil_Driver\cad\RESC1608X342.ipt
- C:\Users\nfitch\Desktop\repos\Imperial\CCMCircuits\CCM_0008_Coil_Driver\cad\RESC1608X343.ipt
- C:\Users\nfitch\Desktop\repos\Imperial\CCMCircuits\CCM_0008_Coil_Driver\cad\RESC1608X344.ipt
- C:\Users\nfitch\Desktop\repos\Imperial\CCMCircuits\CCM_0008_Coil_Driver\cad\RESC1608X345.ipt
- C:\Users\nfitch\Desktop\repos\Imperial\CCMCircuits\CCM_0008_Coil_Driver\cad\RESC1608X346.ipt
- C:\Users\nfitch\Desktop\repos\Imperial\CCMCircuits\CCM_0008_Coil_Driver\cad\RESC1608X347.ipt
- C:\Users\nfitch\Desktop\repos\Imperial\CCMCircuits\CCM_0008_Coil_Driver\cad\RESC1608X348.ipt
- C:\Users\nfitch\Desktop\repos\Imperial\CCMCircuits\CCM_0008_Coil_Driver\cad\RESC1608X349.ipt
- C:\Users\nfitch\Desktop\repos\Imperial\CCMCircuits\CCM_0008_Coil_Driver\cad\RESC1608X350.ipt
- C:\Users\nfitch\Desktop\repos\Imperial\CCMCircuits\CCM_0008_Coil_Driver\cad\RESC1608X351.ipt
- C:\Users\nfitch\Desktop\repos\Imperial\CCMCircuits\CCM_0008_Coil_Driver\cad\RESC1608X352.ipt
- C:\Users\nfitch\Desktop\repos\Imperial\CCMCircuits\CCM_0008_Coil_Driver\cad\RESC1608X353.ipt
- C:\Users\nfitch\Desktop\repos\Imperial\CCMCircuits\CCM_0008_Coil_Driver\cad\RESC1608X354.ipt
- C:\Users\nfitch\Desktop\repos\Imperial\CCMCircuits\CCM_0008_Coil_Driver\cad\RESC1608X355.ipt
- C:\Users\nfitch\Desktop\repos\Imperial\CCMCircuits\CCM_0008_Coil_Driver\cad\RESC1608X356.ipt
- C:\Users\nfitch\Desktop\repos\Imperial\CCMCircuits\CCM_0008_Coil_Driver\cad\RESC1608X357.ipt
- C:\Users\nfitch\Desktop\repos\Imperial\CCMCircuits\CCM_0008_Coil_Driver\cad\RESC1608X358.ipt
- C:\Users\nfitch\Desktop\repos\Imperial\CCMCircuits\CCM_0008_Coil_Driver\cad\RESC1608X359.ipt
- C:\Users\nfitch\Desktop\repos\Imperial\CCMCircuits\CCM_0008_Coil_Driver\cad\RESC1608X360.ipt
- C:\Users\nfitch\Desktop\repos\Imperial\CCMCircuits\CCM_0008_Coil_Driver\cad\RESC1608X361.ipt
- C:\Users\nfitch\Desktop\repos\Imperial\CCMCircuits\CCM_0008_Coil_Driver\cad\RESC1608X362.ipt
- C:\Users\nfitch\Desktop\repos\Imperial\CCMCircuits\CCM_0008_Coil_Driver\cad\RESC1608X363.ipt
- C:\Users\nfitch\Desktop\repos\Imperial\CCMCircuits\CCM_0008_Coil_Driver\cad\RESC1608X364.ipt
- C:\Users\nfitch\Desktop\repos\Imperial\CCMCircuits\CCM_0008_Coil_Driver\cad\RESC1608X365.ipt
- C:\Users\nfitch\Desktop\repos\Imperial\CCMCircuits\CCM_0008_Coil_Driver\cad\RESC1608X366.ipt
- C:\Users\nfitch\Desktop\repos\Imperial\CCMCircuits\CCM_0008_Coil_Driver\cad\RESC1608X367.ipt
- C:\Users\nfitch\Desktop\repos\Imperial\CCMCircuits\CCM_0008_Coil_Driver\cad\RESC1608X368.ipt
- C:\Users\nfitch\Desktop\repos\Imperial\CCMCircuits\CCM_0008_Coil_Driver\cad\RESC1608X369.ipt
- C:\Users\nfitch\Desktop\repos\Imperial\CCMCircuits\CCM_0008_Coil_Driver\cad\RESC1608X370.ipt
- C:\Users\nfitch\Desktop\repos\Imperial\CCMCircuits\CCM_0008_Coil_Driver\cad\RESC1608X371.ipt
- C:\Users\nfitch\Desktop\repos\Imperial\CCMCircuits\CCM_0008_Coil_Driver\cad\RESC1608X372.ipt
- C:\Users\nfitch\Desktop\repos\Imperial\CCMCircuits\CCM_0008_Coil_Driver\cad\RESC1608X373.ipt
- C:\Users\nfitch\Desktop\repos\Imperial\CCMCircuits\CCM_0008_Coil_Driver\cad\RESC1608X374.ipt
- C:\Users\nfitch\Desktop\repos\Imperial\CCMCircuits\CCM_0008_Coil_Driver\cad\RESC1608X375.ipt
- C:\Users\nfitch\Desktop\repos\Imperial\CCMCircuits\CCM_0008_Coil_Driver\cad\RESC1608X376.ipt
- C:\Users\nfitch\Desktop\repos\Imperial\CCMCircuits\CCM_0008_Coil_Driver\cad\RESC1608X377.ipt
- C:\Users\nfitch\Desktop\repos\Imperial\CCMCircuits\CCM_0008_Coil_Driver\cad\RESC1608X378.ipt
- C:\Users\nfitch\Desktop\repos\Imperial\CCMCircuits\CCM_0008_Coil_Driver\cad\RESC1608X379.ipt
- C:\Users\nfitch\Desktop\repos\Imperial\CCMCircuits\CCM_0008_Coil_Driver\cad\RESC1608X380.ipt
- C:\Users\nfitch\Desktop\repos\Imperial\CCMCircuits\CCM_0008_Coil_Driver\cad\RESC1608X381.ipt
- C:\Users\nfitch\Desktop\repos\Imperial\CCMCircuits\CCM_0008_Coil_Driver\cad\RESC1608X382.ipt
- C:\Users\nfitch\Desktop\repos\Imperial\CCMCircuits\CCM_0008_Coil_Driver\cad\RESC1608X383.ipt
- C:\Users\nfitch\Desktop\repos\Imperial\CCMCircuits\CCM_0008_Coil_Driver\cad\RESC1608X384.ipt
- C:\Users\nfitch\Desktop\repos\Imperial\CCMCircuits\CCM_0008_Coil_Driver\cad\RESC1608X385.ipt
- C:\Users\nfitch\Desktop\repos\Imperial\CCMCircuits\CCM_0008_Coil_Driver\cad\RESC1608X386.ipt
- C:\Users\nfitch\Desktop\repos\Imperial\CCMCircuits\CCM_0008_Coil_Driver\cad\RESC1608X387.ipt
- C:\Users\nfitch\Desktop\repos\Imperial\CCMCircuits\CCM_0008_Coil_Driver\cad\RESC1608X388.ipt
- C:\Users\nfitch\Desktop\repos\Imperial\CCMCircuits\CCM_0008_Coil_Driver\cad\RESC1608X389.ipt
- C:\Users\nfitch\Desktop\repos\Imperial\CCMCircuits\CCM_0008_Coil_Driver\cad\RESC1608X390.ipt
- C:\Users\nfitch\Desktop\repos\Imperial\CCMCircuits\CCM_0008_Coil_Driver\cad\RESC1608X391.ipt
- C:\Users\nfitch\Desktop\repos\Imperial\CCMCircuits\CCM_0008_Coil_Driver\cad\RESC1608X392.ipt
- C:\Users\nfitch\Desktop\repos\Imperial\CCMCircuits\CCM_0008_Coil_Driver\cad\RESC1608X393.ipt
- C:\Users\nfitch\Desktop\repos\Imperial\CCMCircuits\CCM_0008_Coil_Driver\cad\RESC1608X394.ipt
- C:\Users\nfitch\Desktop\repos\Imperial\CCMCircuits\CCM_0008_Coil_Driver\cad\RESC1608X395.ipt
- C:\Users\nfitch\Desktop\repos\Imperial\CCMCircuits\CCM_0008_Coil_Driver\cad\RESC1608X396.ipt
- C:\Users\nfitch\Desktop\repos\Imperial\CCMCircuits\CCM_0008_Coil_Driver\cad\RESC1608X397.ipt
- C:\Users\nfitch\Desktop\repos\Imperial\CCMCircuits\CCM_0008_Coil_Driver\cad\RESC1608X398.ipt
- C:\Users\nfitch\Desktop\repos\Imperial\CCMCircuits\CCM_0008_Coil_Driver\cad\RESC1608X399.ipt
- C:\Users\nfitch\Desktop\repos\Imperial\CCMCircuits\CCM_0008_Coil_Driver\cad\RESC1608X400.ipt
- C:\Users\nfitch\Desktop\repos\Imperial\CCMCircuits\CCM_0008_Coil_Driver\cad\RESC1608X401.ipt
- C:\Users\nfitch\Desktop\repos\Imperial\CCMCircuits\CCM_0008_Coil_Driver\cad\RESC1608X402.ipt
- C:\Users\nfitch\Desktop\repos\Imperial\CCMCircuits\CCM_0008_Coil_Driver\cad\RESC1608X403.ipt
- C:\Users\nfitch\Desktop\repos\Imperial\CCMCircuits\CCM_0008_Coil_Driver\cad\RESC1608X404.ipt
- C:\Users\nfitch\Desktop\repos\Imperial\CCMCircuits\CCM_0008_Coil_Driver\cad\RESC1608X405.ipt
- C:\Users\nfitch\Desktop\repos\Imperial\CCMCircuits\CCM_0008_Coil_Driver\cad\RESC1608X406.ipt
- C:\Users\nfitch\Desktop\repos\Imperial\CCMCircuits\CCM_0008_Coil_Driver\cad\RESC1608X407.ipt
- C:\Users\nfitch\Desktop\repos\Imperial\CCMCircuits\CCM_0008_Coil_Driver\cad\RESC1608X408.ipt
- C:\Users\nfitch\Desktop\repos\Imperial\CCMCircuits\CCM_0008_Coil_Driver\cad\RESC1608X409.ipt
- C:\Users\nfitch\Desktop\repos\Imperial\CCMCircuits\CCM_0008_Coil_Driver\cad\RESC1608X410.ipt
- C:\Users\nfitch\Desktop\repos\Imperial\CCMCircuits\CCM_0008_Coil_Driver\cad\RESC1608X411.ipt
- C:\Users\nfitch\Desktop\repos\Imperial\CCMCircuits\CCM_0008_Coil_Driver\cad\RESC1608X412.ipt
- C:\Users\nfitch\Desktop\repos\Imperial\CCMCircuits\CCM_0008_Coil_Driver\cad\RESC1608X413.ipt
- C:\Users\nfitch\Desktop\repos\Imperial\CCMCircuits\CCM_0008_Coil_Driver\cad\RESC1608X414.ipt
- C:\Users\nfitch\Desktop\repos\Imperial\CCMCircuits\CCM_0008_Coil_Driver\cad\RESC1608X415.ipt
- C:\Users\nfitch\Desktop\repos\Imperial\CCMCircuits\CCM_0008_Coil_Driver\cad\RESC1608X416.ipt
- C:\Users\nfitch\Desktop\repos\Imperial\CCMCircuits\CCM_0008_Coil_Driver\cad\RESC1608X417.ipt
- C:\Users\nfitch\Desktop\repos\Imperial\CCMCircuits\CCM_0008_Coil_Driver\cad\RESC1608X418.ipt
- C:\Users\nfitch\Desktop\repos\Imperial\CCMCircuits\CCM_0008_Coil_Driver\cad\RESC1608X419.ipt
- C:\Users\nfitch\Desktop\repos\Imperial\CCMCircuits\CCM_0008_Coil_Driver\cad\RESC1608X420.ipt
- C:\Users\nfitch\Desktop\repos\Imperial\CCMCircuits\CCM_0008_Coil_Driver\cad\RESC1608X421.ipt
- C:\Users\nfitch\Desktop\repos\Imperial\CCMCircuits\CCM_0008_Coil_Driver\cad\RESC1608X422.ipt
- C:\Users\nfitch\Desktop\repos\Imperial\CCMCircuits\CCM_0008_Coil_Driver\cad\RESC1608X423.ipt
- C:\Users\nfitch\Desktop\repos\Imperial\CCMCircuits\CCM_0008_Coil_Driver\cad\RESC1608X424.ipt
- C:\Users\nfitch\Desktop\repos\Imperial\CCMCircuits\CCM_0008_Coil_Driver\cad\RESC1608X425.ipt
- C:\Users\nfitch\Desktop\repos\Imperial\CCMCircuits\CCM_0008_Coil_Driver\cad\RESC1608X426.ipt
- C:\Users\nfitch\Desktop\repos\Imperial\CCMCircuits\CCM_0008_Coil_Driver\cad\RESC1608X427.ipt
- C:\Users\nfitch\Desktop\repos\Imperial\CCMCircuits\CCM_0008_Coil_Driver\cad\RESC1608X428.ipt
- C:\Users\nfitch\Desktop\repos\Imperial\CCMCircuits\CCM_0008_Coil_Driver\cad\RESC1608X429.ipt
- C:\Users\nfitch\Desktop\repos\Imperial\CCMCircuits\CCM_0008_Coil_Driver\cad\RESC1608X430.ipt
- C:\Users\nfitch\Desktop\repos\Imperial\CCMCircuits\CCM_0008_Coil_Driver\cad\RESC1608X431.ipt
- C:\Users\nfitch\Desktop\repos\Imperial\CCMCircuits\CCM_0008_Coil_Driver\cad\RESC1608X432.ipt
- C:\Users\nfitch\Desktop\repos\Imperial\CCMCircuits\CCM_0008_Coil_Driver\cad\RESC1608X433.ipt
- C:\Users\nfitch\Desktop\repos\Imperial\CCMCircuits\CCM_0008_Coil_Driver\cad\RESC1608X434.ipt
- C:\Users\nfitch\Desktop\repos\Imperial\CCMCircuits\CCM_0008_Coil_Driver\cad\RESC1608X435.ipt
- C:\Users\nfitch\Desktop\repos\Imperial\CCMCircuits\CCM_0008_Coil_Driver\cad\RESC1608X436.ipt
- C:\Users\nfitch\Desktop\repos\Imperial\CCMCircuits\CCM_0008_Coil_Driver\cad\RESC1608X437.ipt
- C:\Users\nfitch\Desktop\repos\Imperial\CCMCircuits\CCM_0008_Coil_Driver\cad\RESC1608X438.ipt
- C:\Users\nfitch\Desktop\repos\Imperial\CCMCircuits\CCM_0008_Coil_Driver\cad\RESC1608X439.ipt
- C:\Users\nfitch\Desktop\repos\Imperial\CCMCircuits\CCM_0008_Coil_Driver\cad\RESC1608X440.ipt
- C:\Users\nfitch\Desktop\repos\Imperial\CCMCircuits\CCM_0008_Coil_Driver\cad\RESC1608X441.ipt
- C:\Users\nfitch\Desktop\repos\Imperial\CCMCircuits\CCM_0008_Coil_Driver\cad\RESC1608X442.ipt
- C:\Users\nfitch\Desktop\repos\Imperial\CCMCircuits\CCM_0008_Coil_Driver\cad\RESC1608X443.ipt
- C:\Users\nfitch\Desktop\repos\Imperial\CCMCircuits\CCM_0008_Coil_Driver\cad\RESC1608X444.ipt
- C:\Users\nfitch\Desktop\repos\Imperial\CCMCircuits\CCM_0008_Coil_Driver\cad\RESC1608X445.ipt